# Autodesk Inventor assembly: 歯付きベルト伝達
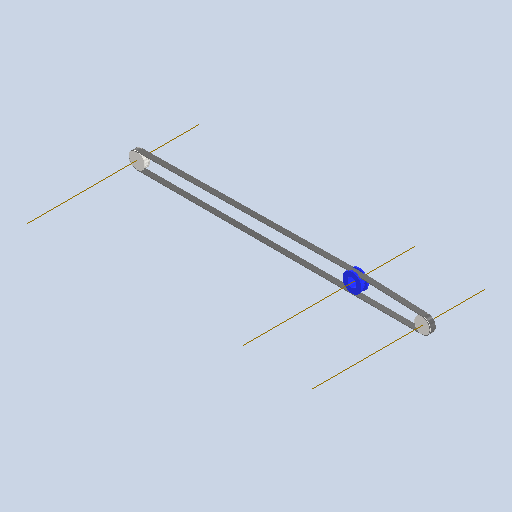
[picture p0: Inventor's stored thumbnail of the model, 512x512]
Saved by Autodesk Inventor 2025.2 (Build 292293000, 293)
## iProperties
ClientObjectVersion: 1
Created: 2025-04-09
Part Number: 歯付きベルト伝達
Document SubType Name: Assembly
Designer: haruy
Author: haruy
## Documents named in this file (5)
- C:\Users\haruy\Documents\ロボコン\NHK2025\cad\nagahisa\dribl\000-dribl-v2\デザイン アクセラレータ\歯付きベルト伝達1.iam
- C:\Users\haruy\Documents\ロボコン\NHK2025\cad\nagahisa\dribl\000-dribl-v2\デザイン アクセラレータ\歯付きベルト1.ipt
- C:\Users\haruy\Documents\ロボコン\NHK2025\cad\nagahisa\dribl\000-dribl-v2\デザイン アクセラレータ\歯付きプーリ11.ipt
- C:\Users\haruy\Documents\ロボコン\NHK2025\cad\nagahisa\dribl\000-dribl-v2\デザイン アクセラレータ\歯付きプーリ21.ipt
- C:\Users\haruy\Documents\ロボコン\NHK2025\cad\nagahisa\dribl\000-dribl-v2\デザイン アクセラレータ\歯付きプーリ31.ipt
## Components (4 placed, 4 different names)
1. 歯付きベルト:1 — フラッシュ:1, メイト:1, メイト:2, フラッシュ:2, メイト:3, メイト:4, フラッシュ:3, メイト:5, メイト:6
2. 歯付きプーリ1:1 — フラッシュ:1, メイト:1, メイト:2, 回転:1, 回転:2
3. 歯付きプーリ2:1 — フラッシュ:2, メイト:3, 回転:1, メイト:4
4. 歯付きプーリ3:1 — フラッシュ:3, メイト:5, 回転:2, メイト:6
## Relationships (11: Mate 6, Flush 3, RelateRotation 2)
- フラッシュ:1 [Flush]: 歯付きベルト:1 ↔ 歯付きプーリ1:1
- メイト:1 [Mate]: 歯付きベルト:1 ↔ 歯付きプーリ1:1
- メイト:2 [Mate]: 歯付きベルト:1 ↔ 歯付きプーリ1:1
- フラッシュ:2 [Flush]: 歯付きベルト:1 ↔ 歯付きプーリ2:1
- メイト:3 [Mate]: 歯付きベルト:1 ↔ 歯付きプーリ2:1
- 回転:1 [RelateRotation] (1 ul): 歯付きプーリ1:1 ↔ 歯付きプーリ2:1
- メイト:4 [Mate]: 歯付きベルト:1 ↔ 歯付きプーリ2:1
- フラッシュ:3 [Flush]: 歯付きベルト:1 ↔ 歯付きプーリ3:1
- メイト:5 [Mate]: 歯付きベルト:1 ↔ 歯付きプーリ3:1
- 回転:2 [RelateRotation] (1 ul): 歯付きプーリ1:1 ↔ 歯付きプーリ3:1
- メイト:6 [Mate]: 歯付きベルト:1 ↔ 歯付きプーリ3:1
